# Autodesk Inventor assembly: Zusammenbau_Schiene
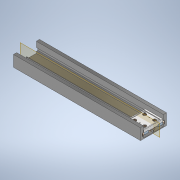
[picture p0: Inventor's stored thumbnail of the model, 180x180]
Saved by Autodesk Inventor 2022 (Build 260153000, 153)
## iProperties
Created: 2022-04-21
Part Number: Zusammenbau_Schiene
Document SubType Name: Assembly
Designer: 123St
Author: 123St
## Documents named in this file (3)
- C:\Users\alexw\Documents\Inventor\Projects\03_CurrentProjects\MasterThesis\PSM_V1_Rillenkugellager\Ueberarbeiteter DaVincikopf\Zusammenbau_Schiene.iam
- C:\Users\alexw\Documents\Inventor\Projects\03_CurrentProjects\MasterThesis\PSM_V1_Rillenkugellager\Ueberarbeiteter DaVincikopf\Zusammenbau.iam
- C:\Users\alexw\Documents\Inventor\Projects\03_CurrentProjects\MasterThesis\PSM_V1_Rillenkugellager\Ueberarbeiteter DaVincikopf\Fuehrungsschiene.ipt
## Components (2 placed, 2 different names)
1. Fuehrungsschiene:1 — Passend:2, Tangential:1, Tangential:2
2. Zusammenbau:1 [sub-assembly] — Passend:2, Tangential:1, Tangential:2
## Relationships (3: Tangent 2, Mate 1)
- Passend:2 [Mate] (7.499 mm): Fuehrungsschiene:1 ↔ Zusammenbau:1
- Tangential:1: Fuehrungsschiene:1 ↔ Zusammenbau:1
- Tangential:2: Fuehrungsschiene:1 ↔ Zusammenbau:1
